# Autodesk Inventor assembly: Updated Frame 2
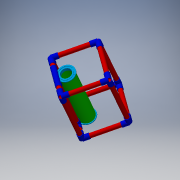
[picture p0: Inventor's stored thumbnail of the model, 180x180]
Saved by Autodesk Inventor 2016 (Build 200138000, 138)
## iProperties
Created: 2017-09-22
Part Number: Updated Frame 2
Document SubType Name: Assembly
Designer: Student
Author: Student
## Documents named in this file (7)
- C:\Users\Student\Documents\Derek Code and Projects\Updated ROV model\Updated Frame 2.iam
- C:\Users\Student\Documents\Derek Code and Projects\Updated ROV model\Updated Frame.iam
- C:\Users\Student\Documents\Derek Code and Projects\CodeBenderCode-master\ROV PVC Pipes\pvc pipe 1in 1ft 1.ipt
- C:\Users\Student\Documents\Derek Code and Projects\Updated ROV model\New Elbow.ipt
- C:\Users\Student\Documents\Derek Code and Projects\CodeBenderCode-master\ROV PVC Pipes\pvc pipe 1in 1.ipt
- C:\Users\Student\Documents\Derek Code and Projects\CodeBenderCode-master\ROV Prototype CAD Models FAILS\Oring Fitting Dome V3.ipt
- C:\Users\Student\Documents\Derek Code and Projects\CodeBenderCode-master\Dome with O-Ring CAD Files\4 inch PVC pipe.ipt
## Components (15 placed, 6 different names)
1. Updated Frame:1 [sub-assembly] — Mate:1, Mate:2, Mate:3, Mate:4, Mate:5, Mate:6, Mate:9, Mate:12, Mate:17, Mate:18, Mate:19, Mate:20, Mate:21, Mate:29, Mate:30
2. pvc pipe 1in 1ft 1:1 — Mate:5, Mate:6
3. pvc pipe 1in 1ft 1:2 — Mate:1, Mate:2
4. pvc pipe 1in 1ft 1:3 — Mate:3, Mate:4
5. New Elbow:1 — Mate:10, Mate:11, Mate:14, Mate:17
6. New Elbow:2 — Mate:10, Mate:11, Mate:12, Mate:13
7. New Elbow:3 — Mate:7, Mate:8, Mate:9, Mate:14, Mate:15, Mate:28
8. New Elbow:4 — Mate:7, Mate:8, Mate:13, Mate:16
9. pvc pipe 1in 1:1 — Mate:16, Mate:27, Mate:30
10. pvc pipe 1in 1:2 — Mate:15, Mate:26, Mate:29
11. pvc pipe 1in 1ft 1:4 — Mate:18, Mate:19
12. pvc pipe 1in 1ft 1:5 — Mate:20, Mate:21
13. Oring Fitting Dome V3:1 — Mate:22, Mate:25, Mate:28
14. Oring Fitting Dome V3:2 — Mate:23, Mate:24
15. 4 inch PVC pipe:1 — Mate:22, Mate:23, Mate:24, Mate:25, Mate:26, Mate:27
## Relationships (30: Mate 30)
- Mate:1: Updated Frame:1 ↔ pvc pipe 1in 1ft 1:2
- Mate:2: Updated Frame:1 ↔ pvc pipe 1in 1ft 1:2
- Mate:3: Updated Frame:1 ↔ pvc pipe 1in 1ft 1:3
- Mate:4: Updated Frame:1 ↔ pvc pipe 1in 1ft 1:3
- Mate:5: Updated Frame:1 ↔ pvc pipe 1in 1ft 1:1
- Mate:6: Updated Frame:1 ↔ pvc pipe 1in 1ft 1:1
- Mate:7: New Elbow:3 ↔ New Elbow:4
- Mate:8: New Elbow:3 ↔ New Elbow:4
- Mate:9: Updated Frame:1 ↔ New Elbow:3
- Mate:10: New Elbow:1 ↔ New Elbow:2
- Mate:11: New Elbow:1 ↔ New Elbow:2
- Mate:12: Updated Frame:1 ↔ New Elbow:2
- Mate:13: New Elbow:2 ↔ New Elbow:4
- Mate:14: New Elbow:1 ↔ New Elbow:3
- Mate:15: New Elbow:3 ↔ pvc pipe 1in 1:2
- Mate:16: New Elbow:4 ↔ pvc pipe 1in 1:1
- Mate:17 (25.4 mm): Updated Frame:1 ↔ New Elbow:1
- Mate:18: Updated Frame:1 ↔ pvc pipe 1in 1ft 1:4
- Mate:19: Updated Frame:1 ↔ pvc pipe 1in 1ft 1:4
- Mate:20: Updated Frame:1 ↔ pvc pipe 1in 1ft 1:5
- Mate:21: Updated Frame:1 ↔ pvc pipe 1in 1ft 1:5
- Mate:22: Oring Fitting Dome V3:1 ↔ 4 inch PVC pipe:1
- Mate:23: Oring Fitting Dome V3:2 ↔ 4 inch PVC pipe:1
- Mate:24: Oring Fitting Dome V3:2 ↔ 4 inch PVC pipe:1
- Mate:25: Oring Fitting Dome V3:1 ↔ 4 inch PVC pipe:1
- Mate:26 (76.2 mm): pvc pipe 1in 1:2 ↔ 4 inch PVC pipe:1
- Mate:27 (76.2 mm): pvc pipe 1in 1:1 ↔ 4 inch PVC pipe:1
- Mate:28 (-38.1 mm): New Elbow:3 ↔ Oring Fitting Dome V3:1
- Mate:29: Updated Frame:1 ↔ pvc pipe 1in 1:2
- Mate:30: Updated Frame:1 ↔ pvc pipe 1in 1:1
